# Autodesk Inventor assembly: ASY MSC 300.2 LEFT BOARD
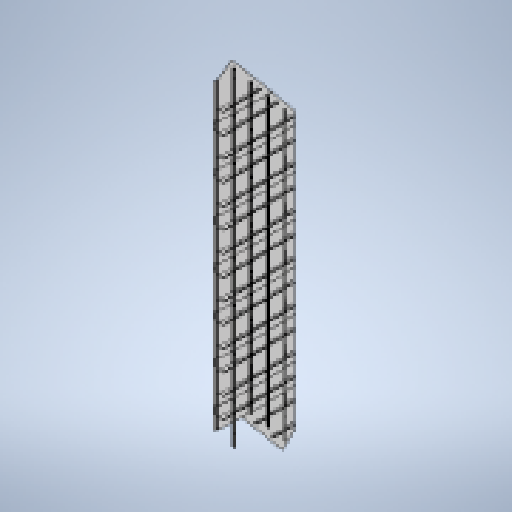
[picture p0: Inventor's stored thumbnail of the model, 512x512]
Saved by Autodesk Inventor 2025.1 (Build 291241020, 241B)
## iProperties
Created: 2024-07-21
Part Number: ASY MSC 300.2 LEFT BOARD
Document SubType Name: Assembly
Designer: pokla
Stock Number: ASY МОО 300.2 левый борт
Mass: 392929 g
Surface Area: 356842 cm^2
Volume: 49116.1 cm^3
Density: 8 g/cm^3
Author: pokla
## Documents named in this file (15)
- C:\Users\user\YandexDisk-badmisterfox\домашниий пк\Inventor\Manturovo\Manturovo_Se-clar\ASY MSC 300.2 LEFT BOARD.iam
- C:\Users\user\YandexDisk-badmisterfox\домашниий пк\Inventor\Manturovo\Manturovo_Se-clar\MSC 340 RIB BOARD.ipt
- C:\Users\user\YandexDisk-badmisterfox\домашниий пк\Inventor\Manturovo\Manturovo_Se-clar\MSC 302 SHEET BOARD MAIN.ipt
- C:\Users\user\YandexDisk-badmisterfox\домашниий пк\Inventor\Manturovo\Manturovo_Se-clar\MSC 301 SHEET LEFT-RIGHT BOARD HIP.ipt
- C:\Users\user\YandexDisk-badmisterfox\домашниий пк\Inventor\Manturovo\Manturovo_Se-clar\MSC 310 SHEET LEFT BOARD WITHERS.ipt
- C:\Users\user\YandexDisk-badmisterfox\домашниий пк\Inventor\Manturovo\Manturovo_Se-clar\MSC 311 SHEET LEFT BOARD FACE.ipt
- C:\Users\user\YandexDisk-badmisterfox\домашниий пк\Inventor\Manturovo\Manturovo_Se-clar\MSC 341 stringer BOARD  #.ipt
- C:\Users\user\YandexDisk-badmisterfox\домашниий пк\Inventor\Manturovo\Manturovo_Se-clar\MSC 342 stringer BOARD  ##.ipt
- C:\Users\user\YandexDisk-badmisterfox\домашниий пк\Inventor\Manturovo\Manturovo_Se-clar\MSC 343 stringer BOARD  ###.ipt
- C:\Users\user\YandexDisk-badmisterfox\домашниий пк\Inventor\Manturovo\Manturovo_Se-clar\MSC 344 stringer BOARD  ####.ipt
- C:\Users\user\YandexDisk-badmisterfox\домашниий пк\Inventor\Manturovo\Manturovo_Se-clar\MSC 313 sheet left board hip.ipt
- C:\Users\user\YandexDisk-badmisterfox\домашниий пк\Inventor\Manturovo\Manturovo_Se-clar\MSC 345 RIB BOARD.ipt
- C:\Users\user\YandexDisk-badmisterfox\домашниий пк\Inventor\Manturovo\Manturovo_Se-clar\MSC 346 RIB BOARD.ipt
- C:\Users\user\YandexDisk-badmisterfox\домашниий пк\Inventor\Manturovo\Manturovo_Se-clar\MSC 347 RIB BOARD.ipt
- C:\Users\user\YandexDisk-badmisterfox\домашниий пк\Inventor\Manturovo\Manturovo_Se-clar\MSC 348 RIB BOARD.ipt
## Components (55 placed, 18 different names)
1. MSC 301 SHEET LEFT-RIGHT BOARD HIP.ipt:1 — Mate:2, Rigid:20, Flush:5, Flush:6, Flush:7, Mate:3, Rigid:51
2. MSC 302 SHEET BOARD MAIN.ipt:1 — Rigid:20, Rigid:21, Flush:8, Tangent:1
3. MSC 302 SHEET BOARD MAIN.ipt:2 — Rigid:21, Rigid:22
4. MSC 302 SHEET BOARD MAIN.ipt:3 — Rigid:22, Rigid:23
5. MSC 302 SHEET BOARD MAIN.ipt:4 — Rigid:23, Rigid:24
6. MSC 302 SHEET BOARD MAIN.ipt:5 — Rigid:24, Rigid:25
7. MSC 310 SHEET LEFT BOARD WITHERS.ipt:1 — Rigid:25, Rigid:26
8. MSC 311 SHEET LEFT BOARD FACE.ipt:1 — Rigid:26
9. MSC 313 sheet left board hip.ipt:1 — Rigid:51
10. MSC 340 RIB BOARD.ipt:1
11. MSC 341 stringer BOARD  #.ipt:1 — Rigid:56
12. MSC 342 stringer BOARD  ##.ipt:1 — Rigid:40, Flush:8, Rigid:55
13. MSC 343 stringer BOARD  ###.ipt:1 — Rigid:41
14. MSC 344 stringer BOARD  ####.ipt:1 — Rigid:42, Rigid:52
15. MSC 340 RIB BOARD.ipt:2
16. MSC 343 stringer BOARD  ###.ipt:2 — Rigid:54
17. MSC 344 stringer BOARD  ####.ipt:2 — Rigid:42, Rigid:57
18. MSC 340 RIB BOARD.ipt:3 — Tangent:1, Mate:3
19. MSC 340 RIB BOARD.ipt:4
20. MSC 340 RIB BOARD.ipt:5 — Rigid:52
21. MSC 340 RIB BOARD.ipt:6 — Rigid:54
22. MSC 342 stringer BOARD  ##:7 — Rigid:55
23. MSC 341 stringer BOARD  #:7 — Rigid:56, Rigid:60, Rigid:61
24. MSC 344 stringer BOARD  ####:8 — Rigid:57
25. MSC 345 RIB BOARD:1 — Rigid:58
26. MSC 346 RIB BOARD:1 — Rigid:59
27. MSC 347 RIB BOARD:1 — Rigid:60
28. MSC 348 RIB BOARD:1 — Rigid:61
29. MSC 340 RIB BOARD.ipt:7 — Rigid:53
30. MSC 340 RIB BOARD.ipt:8
31. MSC 340 RIB BOARD.ipt:9
32. MSC 340 RIB BOARD.ipt:10
33. MSC 340 RIB BOARD.ipt:11
34. MSC 340 RIB BOARD.ipt:12
35. MSC 340 RIB BOARD.ipt:13
36. MSC 344 stringer BOARD  ####.ipt:3 — Rigid:53
37. MSC 343 stringer BOARD  ###.ipt:3 — Rigid:41
38. MSC 342 stringer BOARD  ##.ipt:2 — Rigid:40
39. MSC 341 stringer BOARD  #.ipt:2
40. MSC 344 stringer BOARD  ####:4
41. MSC 343 stringer BOARD  ###:4
42. MSC 342 stringer BOARD  ##:3
43. MSC 341 stringer BOARD  #:3
44. MSC 344 stringer BOARD  ####:5
45. MSC 343 stringer BOARD  ###:5
46. MSC 342 stringer BOARD  ##:4
47. MSC 341 stringer BOARD  #:4
48. MSC 344 stringer BOARD  ####:6 — Rigid:58
49. MSC 343 stringer BOARD  ###:6
50. MSC 342 stringer BOARD  ##:5
51. MSC 341 stringer BOARD  #:5
52. MSC 344 stringer BOARD  ####:7 — Rigid:59
53. MSC 343 stringer BOARD  ###:7
54. MSC 342 stringer BOARD  ##:6
55. MSC 341 stringer BOARD  #:6
## Component patterns: (7 elements, first: MSC 340 RIB BOARD.ipt:7), (5 elements, first: MSC 344 stringer BOARD  ####.ipt:3 + MSC 343 stringer BOARD  ###.ipt:3 + MSC 342 stringer BOARD  ##.ipt:2 + MSC 341 stringer BOARD  #.ipt:2)
## Relationships (38: WeldJoint 31, Flush 4, Mate 2, Tangent 1)
- Mate:2: MSC 301 SHEET LEFT-RIGHT BOARD HIP.ipt:1
- Rigid:20 [WeldJoint]: MSC 301 SHEET LEFT-RIGHT BOARD HIP.ipt:1 ↔ MSC 302 SHEET BOARD MAIN.ipt:1
- Rigid:21 [WeldJoint]: MSC 302 SHEET BOARD MAIN.ipt:1 ↔ MSC 302 SHEET BOARD MAIN.ipt:2
- Rigid:22 [WeldJoint]: MSC 302 SHEET BOARD MAIN.ipt:2 ↔ MSC 302 SHEET BOARD MAIN.ipt:3
- Rigid:23 [WeldJoint]: MSC 302 SHEET BOARD MAIN.ipt:3 ↔ MSC 302 SHEET BOARD MAIN.ipt:4
- Rigid:24 [WeldJoint]: MSC 302 SHEET BOARD MAIN.ipt:4 ↔ MSC 302 SHEET BOARD MAIN.ipt:5
- Rigid:25 [WeldJoint]: MSC 302 SHEET BOARD MAIN.ipt:5 ↔ MSC 310 SHEET LEFT BOARD WITHERS.ipt:1
- Flush:5: MSC 301 SHEET LEFT-RIGHT BOARD HIP.ipt:1
- Flush:6: MSC 301 SHEET LEFT-RIGHT BOARD HIP.ipt:1
- Flush:7: MSC 301 SHEET LEFT-RIGHT BOARD HIP.ipt:1
- Rigid:26 [WeldJoint]: MSC 310 SHEET LEFT BOARD WITHERS.ipt:1 ↔ MSC 311 SHEET LEFT BOARD FACE.ipt:1
- [WeldJoint]: MSC 341 stringer BOARD  #.ipt:1 ↔ MSC 341 stringer BOARD  #.ipt:2
- [WeldJoint]: MSC 343 stringer BOARD  ###.ipt:1 ↔ MSC 343 stringer BOARD  ###.ipt:2
- [WeldJoint]: MSC 344 stringer BOARD  ####.ipt:1 ↔ MSC 344 stringer BOARD  ####.ipt:3
- [WeldJoint] (2 mm): MSC 340 RIB BOARD.ipt:1 ↔ MSC 341 stringer BOARD  #.ipt:2
- [WeldJoint] (2 mm): MSC 341 stringer BOARD  #.ipt:1 ↔ MSC 340 RIB BOARD.ipt:2
- [WeldJoint] (2 mm): MSC 341 stringer BOARD  #.ipt:1 ↔ MSC 340 RIB BOARD.ipt:3
- [WeldJoint] (2 mm): MSC 340 RIB BOARD.ipt:1 ↔ MSC 344 stringer BOARD  ####.ipt:2
- [WeldJoint] (2 mm): MSC 340 RIB BOARD.ipt:1 ↔ MSC 342 stringer BOARD  ##.ipt:1
- [WeldJoint] (2 mm): MSC 340 RIB BOARD.ipt:1 ↔ MSC 343 stringer BOARD  ###.ipt:1
- [WeldJoint] (2 mm): MSC 340 RIB BOARD.ipt:4 ↔ MSC 341 stringer BOARD  #.ipt:2
- Rigid:40 [WeldJoint]: MSC 342 stringer BOARD  ##.ipt:1 ↔ MSC 342 stringer BOARD  ##.ipt:2
- Rigid:41 [WeldJoint]: MSC 343 stringer BOARD  ###.ipt:1 ↔ MSC 343 stringer BOARD  ###.ipt:3
- Rigid:42 [WeldJoint]: MSC 344 stringer BOARD  ####.ipt:1 ↔ MSC 344 stringer BOARD  ####.ipt:2
- Flush:8 (-2 mm): MSC 302 SHEET BOARD MAIN.ipt:1 ↔ MSC 342 stringer BOARD  ##.ipt:1
- Tangent:1: MSC 302 SHEET BOARD MAIN.ipt:1 ↔ MSC 340 RIB BOARD.ipt:3
- Mate:3 (-75 mm): MSC 301 SHEET LEFT-RIGHT BOARD HIP.ipt:1 ↔ MSC 340 RIB BOARD.ipt:3
- Rigid:51 [WeldJoint]: MSC 301 SHEET LEFT-RIGHT BOARD HIP.ipt:1 ↔ MSC 313 sheet left board hip.ipt:1
- Rigid:52 [WeldJoint] (2 mm): MSC 344 stringer BOARD  ####.ipt:1 ↔ MSC 340 RIB BOARD.ipt:5
- Rigid:53 [WeldJoint] (2 mm): MSC 340 RIB BOARD.ipt:7 ↔ MSC 344 stringer BOARD  ####.ipt:3
- Rigid:54 [WeldJoint] (2 mm): MSC 343 stringer BOARD  ###.ipt:2 ↔ MSC 340 RIB BOARD.ipt:6
- Rigid:55 [WeldJoint]: MSC 342 stringer BOARD  ##.ipt:1 ↔ MSC 342 stringer BOARD  ##:7
- Rigid:56 [WeldJoint]: MSC 341 stringer BOARD  #.ipt:1 ↔ MSC 341 stringer BOARD  #:7
- Rigid:57 [WeldJoint]: MSC 344 stringer BOARD  ####.ipt:2 ↔ MSC 344 stringer BOARD  ####:8
- Rigid:58 [WeldJoint] (2 mm): MSC 345 RIB BOARD:1 ↔ MSC 344 stringer BOARD  ####:6
- Rigid:59 [WeldJoint] (2 mm): MSC 346 RIB BOARD:1 ↔ MSC 344 stringer BOARD  ####:7
- Rigid:60 [WeldJoint] (2 mm): MSC 341 stringer BOARD  #:7 ↔ MSC 347 RIB BOARD:1
- Rigid:61 [WeldJoint] (2 mm): MSC 341 stringer BOARD  #:7 ↔ MSC 348 RIB BOARD:1
